# Autodesk Inventor assembly: VolumeKnob
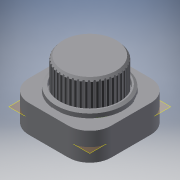
[picture p0: Inventor's stored thumbnail of the model, 180x180]
Saved by Autodesk Inventor 2018 (Build 220112000, 112)
## iProperties
Company: A Company
Created: 2021-11-16
Part Number: VolumeKnob
Material: Generisch
Description: KiCad electronic assembly
Document SubType Name: Assembly
Designer: Markus
Authority: Unknown
Mass: 37.3412 g
Surface Area: 341.907 cm^2
Volume: 29.873 cm^3
Density: 1.25 g/cm^3
Sending System: KiCad to STEP converter
Preprocessor: Open CASCADE STEP processor 6.9
Title: VolumeKnob.step
Author: An Author
## Documents named in this file (11)
- G:\VolumeKnob\3DObjekt\VolumeKnob.iam
- G:\VolumeKnob\3DObjekt\RotaryEncoderV2.iam
- G:\VolumeKnob\3DObjekt\LED_SK6812_PLCC4_5.0x5.0mm_P3.2mm.iam
- G:\VolumeKnob\3DObjekt\Resistor_10K_Ohm_tol1pct_0,25W__07,62.iam
- G:\VolumeKnob\3DObjekt\ArduinoProMicroButtomSoldered.iam
- G:\VolumeKnob\3DObjekt\COMPOUND_2.ipt
- G:\VolumeKnob\3DObjekt\Oberbau.ipt
- G:\VolumeKnob\3DObjekt\Bodenplatte.ipt
- G:\VolumeKnob\3DObjekt\Transfuser.ipt
- G:\VolumeKnob\3DObjekt\Drehregler.ipt
- C:\Users\Markus\Downloads\PAOs4.png
## Components (16 placed, 16 different names)
1. 2 [sub-assembly] — Fluchtend:5
2. 4 [sub-assembly]
3. 6 [sub-assembly]
4. 8 [sub-assembly]
5. 9 [sub-assembly]
6. 10 [sub-assembly]
7. 11 [sub-assembly]
8. 12 [sub-assembly]
9. 13 [sub-assembly]
10. 14 [sub-assembly]
11. 15 [sub-assembly]
12. 16 — Fluchtend:2
13. Oberbau:1 — Fluchtend:2, Fluchtend:4
14. Bodenplatte:1
15. Transfuser:1 — Fluchtend:4
16. Drehregler:1 — Fluchtend:5
## Relationships (3: Flush 3)
- Fluchtend:2 [Flush]: 16 ↔ Oberbau:1
- Fluchtend:4 [Flush]: Oberbau:1 ↔ Transfuser:1
- Fluchtend:5 [Flush]: 2 ↔ Drehregler:1
